# Autodesk Inventor assembly: outer
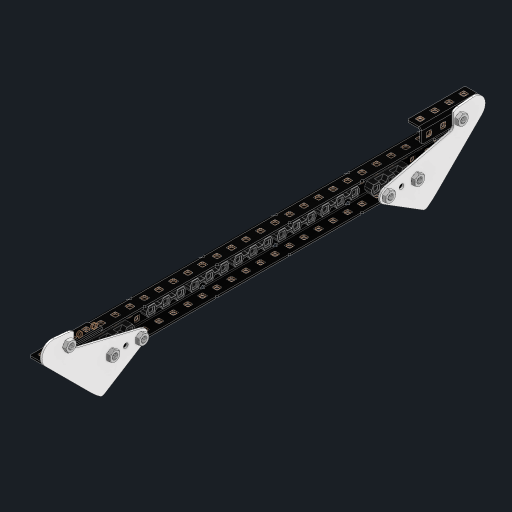
[picture p0: Inventor's stored thumbnail of the model, 512x512]
Saved by Autodesk Inventor 2024 (Build 280153000, 153)
## iProperties
Created: 2024-03-21
Part Number: outer
Document SubType Name: Assembly
Designer: Averey Ku
Author: Averey Ku
## Documents named in this file (9)
- D:\vex_robotics\hardware\cad\infection\chassis\drivebay\outer.iam
- D:\vex_robotics\hardware\cad\VEX-CAD-Inventor-1.41\Motion\Shaft LS\Bearing Flat Low Profile.ipt
- D:\vex_robotics\hardware\cad\VEX-CAD-Inventor-1.41\Structure\Angle\Aluminum 1x1\Alu Angle 1x1x4.ipt
- D:\vex_robotics\hardware\cad\infection\custom_parts\chassis\drivebay\sled.ipt
- D:\vex_robotics\hardware\cad\VEX-CAD-Inventor-1.41\Structure\Hardware\Nut Nylon Thread Forming.ipt
- D:\vex_robotics\hardware\cad\VEX-CAD-Inventor-1.41\Structure\Standoff\Standoff .875.ipt
- D:\vex_robotics\hardware\cad\VEX-CAD-Inventor-1.41\Structure\Standoff.ipt
- D:\vex_robotics\hardware\cad\VEX-CAD-Inventor-1.41\Structure\C Channel\Aluminum 1x2x1\Alu C 1x2x1x26.ipt
- D:\vex_robotics\hardware\cad\infection\custom_parts\chassis\drivebay\sled_l_channel.ipt
## Components (20 placed, 7 different names)
1. Bearing Flat Low Profile:1 — Insert:27, Mate:16, Mate:25
2. Bearing Flat Low Profile:2 — Insert:29, Mate:18
3. Bearing Flat Low Profile:3 — Mate:15, Insert:33, Mate:21
4. Bearing Flat Low Profile:4 — Insert:32, Mate:20
5. Bearing Flat Low Profile:5 — Insert:31, Mate:19
6. Bearing Flat Low Profile:6 — Insert:30
7. Bearing Flat Low Profile:7 — Insert:28, Mate:17
8. sled:1 — Insert:14, Insert:15, Insert:26, Mate:25, Insert:35
9. sled:2 — Mate:15, Insert:17, Insert:18, Insert:24, Insert:25
10. Nut Nylon Thread Forming:2 — Insert:26
11. Nut Nylon Thread Forming:3 — Insert:15
12. Nut Nylon Thread Forming:4 — Insert:14
13. Alu Angle 1x1x4:2 — Insert:24, Mate:22, Mate:23
14. Nut Nylon Thread Forming:5 — Insert:17
15. Nut Nylon Thread Forming:7 — Insert:18
16. Nut Nylon Thread Forming:8 — Insert:25
17. Standoff .875:1
18. Standoff .875:2
19. Alu C 1x2x1x26:1 — Insert:27, Mate:16, Insert:28, Mate:17, Insert:29, Mate:18, Insert:30, Insert:31, Mate:19, Insert:32, Mate:20, Insert:33, Mate:21, Mate:22, Mate:23, Insert:34, Mate:26
20. sled_l_channel:1 — Insert:34, Mate:26, Insert:35
## Relationships (27: Insert 16, Mate 11)
- Insert:14: sled:1 ↔ Nut Nylon Thread Forming:4
- Insert:15: sled:1 ↔ Nut Nylon Thread Forming:3
- Mate:15: Bearing Flat Low Profile:3 ↔ sled:2
- Insert:17: sled:2 ↔ Nut Nylon Thread Forming:5
- Insert:18: sled:2 ↔ Nut Nylon Thread Forming:7
- Insert:24: sled:2 ↔ Alu Angle 1x1x4:2
- Insert:25: sled:2 ↔ Nut Nylon Thread Forming:8
- Insert:26: sled:1 ↔ Nut Nylon Thread Forming:2
- Insert:27: Bearing Flat Low Profile:1 ↔ Alu C 1x2x1x26:1
- Mate:16: Bearing Flat Low Profile:1 ↔ Alu C 1x2x1x26:1
- Insert:28: Bearing Flat Low Profile:7 ↔ Alu C 1x2x1x26:1
- Mate:17: Bearing Flat Low Profile:7 ↔ Alu C 1x2x1x26:1
- Insert:29: Bearing Flat Low Profile:2 ↔ Alu C 1x2x1x26:1
- Mate:18: Bearing Flat Low Profile:2 ↔ Alu C 1x2x1x26:1
- Insert:30: Bearing Flat Low Profile:6 ↔ Alu C 1x2x1x26:1
- Insert:31: Bearing Flat Low Profile:5 ↔ Alu C 1x2x1x26:1
- Mate:19: Bearing Flat Low Profile:5 ↔ Alu C 1x2x1x26:1
- Insert:32: Bearing Flat Low Profile:4 ↔ Alu C 1x2x1x26:1
- Mate:20: Bearing Flat Low Profile:4 ↔ Alu C 1x2x1x26:1
- Insert:33: Bearing Flat Low Profile:3 ↔ Alu C 1x2x1x26:1
- Mate:21: Bearing Flat Low Profile:3 ↔ Alu C 1x2x1x26:1
- Mate:22: Alu Angle 1x1x4:2 ↔ Alu C 1x2x1x26:1
- Mate:23: Alu Angle 1x1x4:2 ↔ Alu C 1x2x1x26:1
- Mate:25: Bearing Flat Low Profile:1 ↔ sled:1
- Insert:34: Alu C 1x2x1x26:1 ↔ sled_l_channel:1
- Mate:26: Alu C 1x2x1x26:1 ↔ sled_l_channel:1
- Insert:35: sled:1 ↔ sled_l_channel:1
